# Autodesk Inventor assembly: GFRP_T2_04
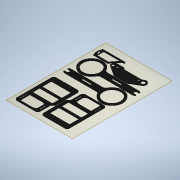
[picture p0: Inventor's stored thumbnail of the model, 180x180]
Saved by Autodesk Inventor 2020 (Build 240168000, 168)
## iProperties
Created: 2021-08-27
Part Number: GFRP_T2_04
Document SubType Name: Assembly
Designer: Masato
Author: Masato
## Documents named in this file (6)
- C:\Inventor\SUSTAINA-OP_0317_01\Cam\GFRP_T2_04.iam
- C:\Inventor\SUSTAINA-OP_0317_01\Cam\DisposableBoard.ipt
- C:\Inventor\SUSTAINA-OP_0317_01\UpperBody\Trunk\Trunk_upper_side_frame.ipt
- C:\Inventor\SUSTAINA-OP_0317_01\UpperBody\Arm\ForeArm_outside_frame.ipt
- C:\Inventor\SUSTAINA-OP_0317_01\LowerBody\Link\FrontLink_frame.ipt
- C:\Inventor\SUSTAINA-OP_0317_01\UpperBody\Arm\UpperArm_side_frame.ipt
## Components (7 placed, 5 different names)
1. DisposableBoard:1 — メイト:2, メイト:1, フラッシュ:1, フラッシュ:2, メイト:4, メイト:5, フラッシュ:3, フラッシュ:4, メイト:7, メイト:8, 正接:2, 正接:3, 角度:1, 正接:6, メイト:9, メイト:10, フラッシュ:6
2. Trunk_upper_side_frame:1 — メイト:4, フラッシュ:3, フラッシュ:4, フラッシュ:5, メイト:6
3. Trunk_upper_side_frame:2 — メイト:5, フラッシュ:5, メイト:6, 正接:1
4. ForeArm_outside_frame:1 — メイト:7, 正接:1, 正接:2, 正接:3, 正接:4, 正接:5
5. ForeArm_outside_frame:2 — メイト:8, 角度:1, 正接:4, 正接:5, 正接:6, 正接:7, メイト:11
6. FrontLink_frame:1 — メイト:10, メイト:11, 正接:8
7. UpperArm_side_frame:1 — メイト:9, 正接:7, フラッシュ:6, 正接:8
## Relationships (25: Mate 10, Tangent 8, Flush 6, Angle 1)
- メイト:2 [Mate]: DisposableBoard:1
- メイト:1 [Mate]: DisposableBoard:1
- フラッシュ:1 [Flush]: DisposableBoard:1
- フラッシュ:2 [Flush]: DisposableBoard:1
- メイト:4 [Mate]: DisposableBoard:1 ↔ Trunk_upper_side_frame:1
- メイト:5 [Mate]: DisposableBoard:1 ↔ Trunk_upper_side_frame:2
- フラッシュ:3 [Flush] (1.5 mm): DisposableBoard:1 ↔ Trunk_upper_side_frame:1
- フラッシュ:4 [Flush] (1.5 mm): DisposableBoard:1 ↔ Trunk_upper_side_frame:1
- フラッシュ:5 [Flush]: Trunk_upper_side_frame:1 ↔ Trunk_upper_side_frame:2
- メイト:6 [Mate] (2.5 mm): Trunk_upper_side_frame:1 ↔ Trunk_upper_side_frame:2
- メイト:7 [Mate]: DisposableBoard:1 ↔ ForeArm_outside_frame:1
- メイト:8 [Mate]: DisposableBoard:1 ↔ ForeArm_outside_frame:2
- 正接:1 [Tangent] (2.5 mm): Trunk_upper_side_frame:2 ↔ ForeArm_outside_frame:1
- 正接:2 [Tangent] (2.5 mm): DisposableBoard:1 ↔ ForeArm_outside_frame:1
- 正接:3 [Tangent] (2.5 mm): DisposableBoard:1 ↔ ForeArm_outside_frame:1
- 角度:1 [Angle] (90 deg): DisposableBoard:1 ↔ ForeArm_outside_frame:2
- 正接:4 [Tangent] (2.5 mm): ForeArm_outside_frame:1 ↔ ForeArm_outside_frame:2
- 正接:5 [Tangent] (2.5 mm): ForeArm_outside_frame:1 ↔ ForeArm_outside_frame:2
- 正接:6 [Tangent] (2.5 mm): DisposableBoard:1 ↔ ForeArm_outside_frame:2
- メイト:9 [Mate]: DisposableBoard:1 ↔ UpperArm_side_frame:1
- メイト:10 [Mate]: DisposableBoard:1 ↔ FrontLink_frame:1
- 正接:7 [Tangent] (2.5 mm): ForeArm_outside_frame:2 ↔ UpperArm_side_frame:1
- フラッシュ:6 [Flush] (2 mm): DisposableBoard:1 ↔ UpperArm_side_frame:1
- メイト:11 [Mate] (2.5 mm): ForeArm_outside_frame:2 ↔ FrontLink_frame:1
- 正接:8 [Tangent] (2.5 mm): FrontLink_frame:1 ↔ UpperArm_side_frame:1
